# Autodesk Inventor assembly: total assemble
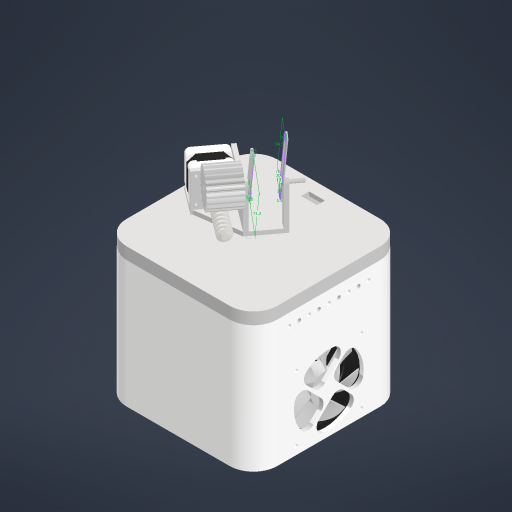
[picture p0: Inventor's stored thumbnail of the model, 512x512]
Saved by Autodesk Inventor 2024.2 (Build 282272000, 272)
## iProperties
Created: 2023-07-11
Part Number: total assemble
Document SubType Name: Assembly
Designer: 6gioc
Author: 6gioc
## Documents named in this file (15)
- C:\Users\6gioc\OneDrive\AAST\PART\AAST Main\total assemble.iam
- C:\Users\6gioc\OneDrive\AAST\PART\AAST Main\bottom part v2.ipt
- C:\Users\6gioc\OneDrive\AAST\PART\AAST Main\smps.ipt
- C:\Users\6gioc\OneDrive\AAST\PART\AAST Main\FAN.iam
- C:\Users\6gioc\OneDrive\AAST\PART\AAST Main\outlet.ipt
- C:\Users\6gioc\OneDrive\AAST\PART\AAST Main\smps power crossbar.ipt
- C:\Users\6gioc\OneDrive\AAST\PART\AAST Main\stepmotor v1.ipt
- C:\Users\6gioc\OneDrive\AAST\PART\AAST Main\horizental blade.ipt
- C:\Users\6gioc\OneDrive\AAST\PART\AAST Main\wind blade.ipt
- C:\Users\6gioc\OneDrive\AAST\PART\AAST Main\Raspberry Pi 4 Model B\Raspberry Pi 4 Model B.iam
- C:\Users\6gioc\OneDrive\AAST\PART\AAST Main\pcb.ipt
- C:\Users\6gioc\OneDrive\AAST\PART\AAST Main\top.ipt
- C:\Users\6gioc\OneDrive\AAST\PART\AAST Main\worm.iam
- C:\Users\6gioc\OneDrive\AAST\PART\AAST Main\gun assemble v1.iam
- C:\Users\6gioc\OneDrive\AAST\PART\AAST Main\40mm_gear_hexagon.iam
## Components (17 placed, 14 different names)
1. bottom part v2:1 — 강체:1, 강체:2, 강체:3, 강체:4, 강체:5, 강체:9, 강체:11, 강체:14
2. smps:1 — 강체:5, 강체:6, 회전:1
3. smps:2 — 강체:4, 회전:2
4. FAN:1 [sub-assembly] — 강체:1
5. FAN:2 [sub-assembly] — 강체:2
6. outlet:1 — 강체:3
7. smps power crossbar:1 — 강체:6, 강체:8, 강체:13, 강체:14
8. stepmotor v1:1 — 강체:10, 회전:3
9. horizental blade:1 — 강체:13
10. wind blade:1 — 회전:1
11. wind blade:2 — 회전:2
12. Raspberry Pi 4 Model B:1 [sub-assembly] — 강체:8
13. pcb:1 — 강체:9
14. top:1 — 강체:10, 강체:11, 회전:4
15. worm:1 [sub-assembly] — 회전:3, 회전:1
16. gun assemble v1:1 [sub-assembly] — 회전:4, 강체:12, 회전:1
17. 40mm_gear_hexagon:1 [sub-assembly] — 강체:12
## Relationships (18: WeldJoint 13, RevoluteJoint 4, RelateRotation 1)
- 강체:1 [WeldJoint]: bottom part v2:1 ↔ FAN:1
- 강체:2 [WeldJoint]: bottom part v2:1 ↔ FAN:2
- 강체:3 [WeldJoint]: bottom part v2:1 ↔ outlet:1
- 강체:4 [WeldJoint]: bottom part v2:1 ↔ smps:2
- 강체:5 [WeldJoint]: bottom part v2:1 ↔ smps:1
- 강체:6 [WeldJoint]: smps:1 ↔ smps power crossbar:1
- 회전:1 [RevoluteJoint]: smps:1 ↔ wind blade:1
- 회전:2 [RevoluteJoint]: smps:2 ↔ wind blade:2
- 강체:8 [WeldJoint]: smps power crossbar:1 ↔ Raspberry Pi 4 Model B:1
- 강체:9 [WeldJoint]: bottom part v2:1 ↔ pcb:1
- 강체:10 [WeldJoint]: stepmotor v1:1 ↔ top:1
- 강체:11 [WeldJoint]: bottom part v2:1 ↔ top:1
- 회전:3 [RevoluteJoint]: stepmotor v1:1 ↔ worm:1
- 회전:4 [RevoluteJoint]: top:1 ↔ gun assemble v1:1
- 강체:12 [WeldJoint]: gun assemble v1:1 ↔ 40mm_gear_hexagon:1
- 회전:1 [RelateRotation] (-0.05 ul): worm:1 ↔ gun assemble v1:1
- 강체:13 [WeldJoint]: smps power crossbar:1 ↔ horizental blade:1
- 강체:14 [WeldJoint]: bottom part v2:1 ↔ smps power crossbar:1
